# Autodesk Inventor assembly: PSUMount
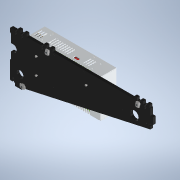
[picture p0: Inventor's stored thumbnail of the model, 180x180]
Saved by Autodesk Inventor 2020.2 (Build 242310000, 310)
## iProperties
Created: 2020-08-24
Part Number: PSUMount
Document SubType Name: Assembly
Designer: JK
Author: JK
## Documents named in this file (6)
- C:\Users\JK\Documents\Inventor\Anet Upgrade\PSUMount.iam
- C:\Users\JK\Documents\Inventor\Anet Upgrade\acrylicframepart.ipt
- C:\Users\JK\Documents\Inventor\Anet Upgrade\T_Slot_Nut_Dropin_3030m5ipt.ipt
- C:\Users\JK\Documents\Inventor\Anet Upgrade\M5x15BoltFlatHead.ipt
- C:\Users\JK\Documents\Inventor\Anet Upgrade\Power Supply 12 V.iam
- C:\Users\JK\Documents\Inventor\Anet Upgrade\M3X15.ipt
## Components (11 placed, 5 different names)
1. acrylicframepart:1 — Mate:1, Mate:2, Mate:3, Angle:1, Mate:7, Mate:8, Mate:9, Mate:10, Angle:4, Mate:11, Mate:12, Mate:13, Mate:14
2. M5x15BoltFlatHead:1 — Mate:1, Mate:6, Mate:7, Flush:1
3. M5x15BoltFlatHead:2 — Mate:2, Mate:4, Flush:1, Flush:2
4. M5x15BoltFlatHead:3 — Mate:3, Mate:5, Flush:2
5. T_Slot_Nut_Dropin_3030m5ipt:1 — Mate:4, Angle:2, Angle:3, Flush:3, Flush:4
6. T_Slot_Nut_Dropin_3030m5ipt:2 — Mate:5, Angle:3, Flush:4
7. T_Slot_Nut_Dropin_3030m5ipt:3 — Mate:6, Angle:1, Angle:2, Mate:8, Flush:3
8. Power Supply 12 V:1 [sub-assembly] — Mate:9, Mate:10, Angle:4
9. Unbrako Hex Socket Cap - Metric M3 x 25:1 — Mate:12, Flush:5
10. Unbrako Hex Socket Cap - Metric M3 x 25:2 — Mate:13, Flush:6, Mate:14
11. Unbrako Hex Socket Cap - Metric M3 x 25:3 — Mate:11, Flush:5, Flush:6
## Relationships (24: Mate 14, Flush 6, Angle 4)
- Mate:1: acrylicframepart:1 ↔ M5x15BoltFlatHead:1
- Mate:2: acrylicframepart:1 ↔ M5x15BoltFlatHead:2
- Mate:3: acrylicframepart:1 ↔ M5x15BoltFlatHead:3
- Mate:4: M5x15BoltFlatHead:2 ↔ T_Slot_Nut_Dropin_3030m5ipt:1
- Mate:5: M5x15BoltFlatHead:3 ↔ T_Slot_Nut_Dropin_3030m5ipt:2
- Mate:6: M5x15BoltFlatHead:1 ↔ T_Slot_Nut_Dropin_3030m5ipt:3
- Angle:1 (0 deg): acrylicframepart:1 ↔ T_Slot_Nut_Dropin_3030m5ipt:3
- Angle:2 (0 deg): T_Slot_Nut_Dropin_3030m5ipt:1 ↔ T_Slot_Nut_Dropin_3030m5ipt:3
- Angle:3 (90 deg): T_Slot_Nut_Dropin_3030m5ipt:1 ↔ T_Slot_Nut_Dropin_3030m5ipt:2
- Mate:7: acrylicframepart:1 ↔ M5x15BoltFlatHead:1
- Flush:1: M5x15BoltFlatHead:1 ↔ M5x15BoltFlatHead:2
- Flush:2: M5x15BoltFlatHead:2 ↔ M5x15BoltFlatHead:3
- Mate:8: acrylicframepart:1 ↔ T_Slot_Nut_Dropin_3030m5ipt:3
- Flush:3: T_Slot_Nut_Dropin_3030m5ipt:1 ↔ T_Slot_Nut_Dropin_3030m5ipt:3
- Flush:4: T_Slot_Nut_Dropin_3030m5ipt:1 ↔ T_Slot_Nut_Dropin_3030m5ipt:2
- Mate:9: acrylicframepart:1 ↔ Power Supply 12 V:1
- Mate:10: acrylicframepart:1 ↔ Power Supply 12 V:1
- Angle:4 (0 deg): acrylicframepart:1 ↔ Power Supply 12 V:1
- Mate:11: acrylicframepart:1 ↔ Unbrako Hex Socket Cap - Metric M3 x 25:3
- Mate:12: acrylicframepart:1 ↔ Unbrako Hex Socket Cap - Metric M3 x 25:1
- Mate:13: acrylicframepart:1 ↔ Unbrako Hex Socket Cap - Metric M3 x 25:2
- Flush:5: Unbrako Hex Socket Cap - Metric M3 x 25:1 ↔ Unbrako Hex Socket Cap - Metric M3 x 25:3
- Flush:6: Unbrako Hex Socket Cap - Metric M3 x 25:2 ↔ Unbrako Hex Socket Cap - Metric M3 x 25:3
- Mate:14: acrylicframepart:1 ↔ Unbrako Hex Socket Cap - Metric M3 x 25:2
